# Autodesk Inventor assembly: Top rollers
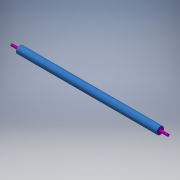
[picture p0: Inventor's stored thumbnail of the model, 180x180]
Saved by Autodesk Inventor 2017 (Build 210142000, 142)
## iProperties
Created: 2017-01-17
Part Number: Top rollers
Document SubType Name: Assembly
Designer: Ben
Author: Ben
## Documents named in this file (3)
- C:\Users\Ben\Desktop\Projects\2017 Robot\Ball Intake\Top rollers.iam
- C:\Users\Ben\Desktop\Projects\2017 Robot\Ball Intake\1in PVC Roller.ipt
- C:\Users\Ben\Desktop\Projects\2017 Robot\Ball Intake\Long roller plug.ipt
## Components (3 placed, 2 different names)
1. 1in PVC Roller:1 — Insert:1, Insert:2
2. Long roller plug:1 — Insert:1
3. Long roller plug:2 — Insert:2
## Relationships (2: Insert 2)
- Insert:1: 1in PVC Roller:1 ↔ Long roller plug:1
- Insert:2: 1in PVC Roller:1 ↔ Long roller plug:2
